# Autodesk Inventor assembly: AE_100MM_ASSEM
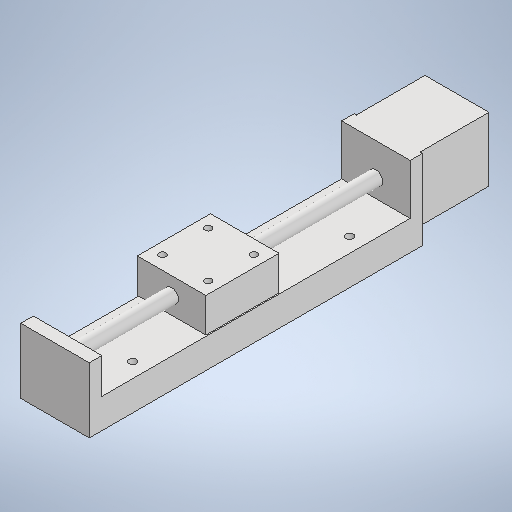
[picture p0: Inventor's stored thumbnail of the model, 512x512]
Saved by Autodesk Inventor 2025.2 (Build 292293000, 293)
## iProperties
Created: 2026-02-09
Part Number: AE_100MM_ASSEM
Document SubType Name: Assembly
Designer: composite
Author: composite
## Documents named in this file (3)
- H:\01-Members Space\Sam Munro\Extrusion Printer\Printer V2\PRINTESS FILES\AE_100MM_ASSEM.iam
- H:\01-Members Space\Sam Munro\Extrusion Printer\Printer V2\PRINTESS FILES\AE_100MM_STAGE.ipt
- H:\01-Members Space\Sam Munro\Extrusion Printer\Printer V2\PRINTESS FILES\AE_MOVING_STAGE.ipt
## Components (2 placed, 2 different names)
1. AE_100MM_STAGE:1 — Mate:1, Angle:1
2. AE_MOVING_STAGE:1 — Mate:1, Angle:1
## Relationships (2: Mate 1, Angle 1)
- Mate:1: AE_100MM_STAGE:1 ↔ AE_MOVING_STAGE:1
- Angle:1 (0 deg): AE_100MM_STAGE:1 ↔ AE_MOVING_STAGE:1
